# Autodesk Inventor assembly: motor&arm_MIR1_CPY
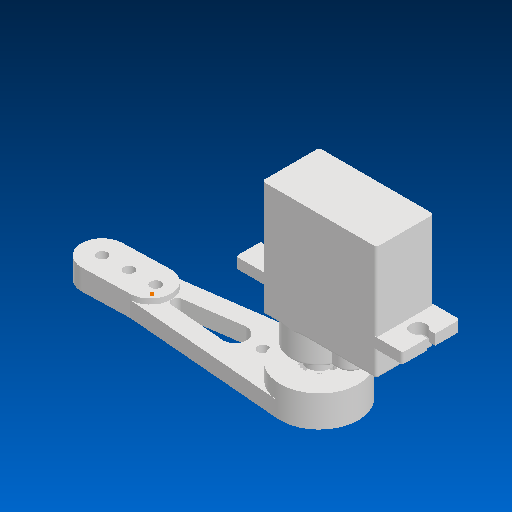
[picture p0: Inventor's stored thumbnail of the model, 512x512]
Saved by Autodesk Inventor 2020.2 (Build 242310000, 310)
## iProperties
Created: 2020-02-16
Part Number: motor&arm_MIR1_CPY
Document SubType Name: Assembly
Designer: Yash
Author: Yash
## Documents named in this file (3)
- E:\KLE\Engineering Exploration\Model\motor&arm_MIR1_CPY.iam
- E:\KLE\Engineering Exploration\Model\Servo Motor SG90_MIR1_CPY.ipt
- E:\KLE\Engineering Exploration\Model\servo arm_MIR1_CPY.ipt
## Components (2 placed, 2 different names)
1. Servo Motor SG90_MIR1_CPY:1 — Insert:1
2. servo arm_MIR1_CPY:1 — Insert:1
## Relationships (1: Insert 1)
- Insert:1: Servo Motor SG90_MIR1_CPY:1 ↔ servo arm_MIR1_CPY:1
